# Autodesk Inventor assembly: Assembly1
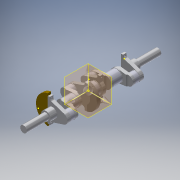
[picture p0: Inventor's stored thumbnail of the model, 180x180]
Saved by Autodesk Inventor 2019 (Build 230136000, 136)
## iProperties
Created: 2019-06-29
Part Number: Assembly1
Document SubType Name: Assembly
Designer: usuario
Author: usuario
## Documents named in this file (5)
- E:\OSCAR\UNAL\6to SEMESTRE\Principios de dinámica\Proyectos\Proyecto 2\Mio\Assembly1.iam
- E:\OSCAR\UNAL\6to SEMESTRE\Principios de dinámica\Proyectos\Proyecto 2\Mio\cigueñal.ipt
- E:\OSCAR\UNAL\6to SEMESTRE\Principios de dinámica\Proyectos\Proyecto 2\Mio\Contrapeso2.ipt
- E:\OSCAR\UNAL\6to SEMESTRE\Principios de dinámica\Proyectos\Proyecto 2\Mio\ContrapesoGrande1.ipt
- E:\OSCAR\UNAL\6to SEMESTRE\Principios de dinámica\Proyectos\Proyecto 2\Mio\Pasador.ipt
## Components (4 placed, 4 different names)
1. cigueñal:1 — Rigid:1, Rigid:2
2. ContrapesoGrande1:1 — Rigid:1, Insert:1
3. Contrapeso2:1 — Rigid:2
4. Pasador:1 — Insert:1
## Relationships (3: WeldJoint 2, Insert 1)
- Rigid:1 [WeldJoint]: cigueñal:1 ↔ ContrapesoGrande1:1
- Rigid:2 [WeldJoint]: cigueñal:1 ↔ Contrapeso2:1
- Insert:1 (-17 mm): ContrapesoGrande1:1 ↔ Pasador:1
